# Autodesk Inventor assembly: SHOT_0_000_PivotAssembly
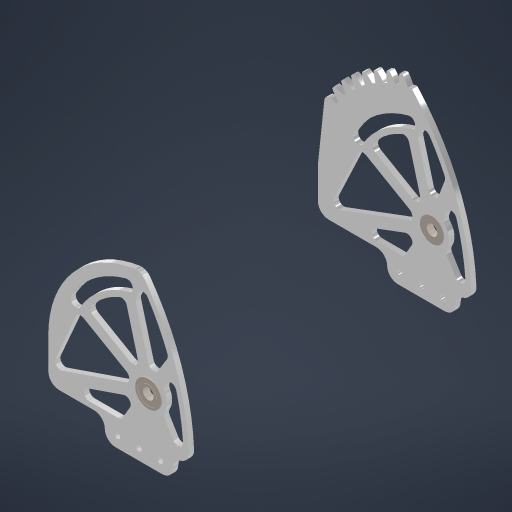
[picture p0: Inventor's stored thumbnail of the model, 512x512]
Saved by Autodesk Inventor 2024.2 (Build 282272000, 272)
## iProperties
Created: 2024-08-07
Part Number: SHOT_0_000_PivotAssembly
Document SubType Name: Assembly
Designer: Bryan
Mass: 708.017 g
Surface Area: 1048.32 cm^2
Volume: 246.247 cm^3
Density: 2.87523 g/cm^3
Author: Bryan
## Documents named in this file (4)
- C:\Users\bobsb\OneDrive\Documents\GitHub\1622-2024-Summer-CAD-A-Thon\Shooter\SHOT_0_000_PivotAssembly.iam
- C:\Users\bobsb\OneDrive\Documents\GitHub\1622-2024-Summer-CAD-A-Thon\Shooter\SHOT_0_001_PivotGear.ipt
- C:\Users\bobsb\OneDrive\Documents\GitHub\1622-2024-Summer-CAD-A-Thon\Shooter\SHOT_0_002_PivotPlate.ipt
- C:\Users\bobsb\OneDrive\Documents\GitHub\1622-2024-Summer-CAD-A-Thon\COTS Library\Motion\Bearings\COTS_WCP-0781_0.5ODCircularFlangedBearing.ipt
## Components (4 placed, 3 different names)
1. SHOT_0_001_PivotGear:1 — Mate:1, Mate:3, Mate:4, Mate:7, Mate:8
2. SHOT_0_002_PivotPlate:1 — Mate:1, Mate:3, Mate:4, Mate:5, Mate:6
3. COTS_WCP-0781_0.5ODCircularFlangedBearing:1 — Mate:5, Mate:6
4. COTS_WCP-0781_0.5ODCircularFlangedBearing:2 — Mate:7, Mate:8
## Relationships (7: Mate 7)
- Mate:1: SHOT_0_001_PivotGear:1 ↔ SHOT_0_002_PivotPlate:1
- Mate:3 (330.2 mm): SHOT_0_001_PivotGear:1 ↔ SHOT_0_002_PivotPlate:1
- Mate:4: SHOT_0_001_PivotGear:1 ↔ SHOT_0_002_PivotPlate:1
- Mate:5: SHOT_0_002_PivotPlate:1 ↔ COTS_WCP-0781_0.5ODCircularFlangedBearing:1
- Mate:6: SHOT_0_002_PivotPlate:1 ↔ COTS_WCP-0781_0.5ODCircularFlangedBearing:1
- Mate:7: SHOT_0_001_PivotGear:1 ↔ COTS_WCP-0781_0.5ODCircularFlangedBearing:2
- Mate:8: SHOT_0_001_PivotGear:1 ↔ COTS_WCP-0781_0.5ODCircularFlangedBearing:2
